# Autodesk Inventor assembly: Sestava
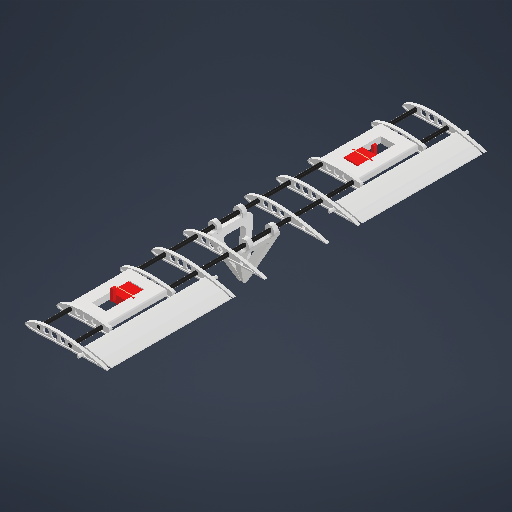
[picture p0: Inventor's stored thumbnail of the model, 512x512]
Saved by Autodesk Inventor 2026 (Build 300175050, 175E)
## iProperties
Created: 2026-02-21
Part Number: Sestava
Document SubType Name: Assembly
Designer: marti
Mass: 312.301 g
Surface Area: 1695.85 cm^2
Volume: 283.461 cm^3
Density: 1.10174 g/cm^3
Author: marti
## Documents named in this file (9)
- F:\Ročníkovka\RP_Svitek\3d model\lepší\Sestava.iam
- F:\Ročníkovka\RP_Svitek\3d model\lepší\tyč.ipt
- F:\Ročníkovka\RP_Svitek\3d model\lepší\Profil.ipt
- F:\Ročníkovka\RP_Svitek\3d model\lepší\NOAileron.ipt
- F:\Ročníkovka\RP_Svitek\3d model\lepší\Aileronn.ipt
- F:\Ročníkovka\RP_Svitek\3d model\lepší\vetrovaniig.ipt
- F:\Ročníkovka\RP_Svitek\3d model\lepší\trojúhleník.ipt
- F:\Ročníkovka\RP_Svitek\3d model\lepší\SERVO držák.ipt
- F:\Ročníkovka\RP_Svitek\3d model\lepší\Servo.ipt
## Components (21 placed, 8 different names)
1. tyč:1 — Proti sobě:1, Stejný směr:1, Proti sobě:2, Proti sobě:3, Proti sobě:4, Proti sobě:8, Proti sobě:10, Proti sobě:12, Proti sobě:14, Proti sobě:17, Stejný směr:2, Proti sobě:22, Proti sobě:27, Proti sobě:29, Proti sobě:31, Proti sobě:43, Proti sobě:47, Proti sobě:53, Proti sobě:54
2. tyč:2 — Proti sobě:4, Proti sobě:5, Proti sobě:6, Proti sobě:7, Proti sobě:9, Proti sobě:11, Proti sobě:13, Proti sobě:15, Proti sobě:18, Stejný směr:2, Stejný směr:3, Proti sobě:23, Stejný směr:4, Proti sobě:28, Proti sobě:30, Proti sobě:32, Proti sobě:44, Proti sobě:46, Proti sobě:51, Stejný směr:14
3. Profil:1 — Proti sobě:2, Proti sobě:6, Stejný směr:4, Proti sobě:24, Proti sobě:25, Stejný směr:5
4. Profil:2 — Proti sobě:3, Proti sobě:7, Proti sobě:16, Proti sobě:19, Proti sobě:20, Stejný směr:3, Stejný směr:9
5. NOAileron:1 — Proti sobě:8, Proti sobě:9, Stejný směr:5, Stejný směr:6
6. NOAileron:2 — Proti sobě:10, Proti sobě:11, Stejný směr:6, Stejný směr:7, Proti sobě:45
7. NOAileron:3 — Proti sobě:14, Proti sobě:15, Stejný směr:9, Stejný směr:10
8. NOAileron:4 — Proti sobě:12, Proti sobě:13, Stejný směr:10, Stejný směr:11, Proti sobě:48
9. Profil:3 — Proti sobě:22, Proti sobě:23, Proti sobě:26, Stejný směr:7, Stejný směr:8
10. Profil:4 — Proti sobě:17, Proti sobě:18, Proti sobě:21, Stejný směr:11, Stejný směr:12
11. Aileronn:1 — Proti sobě:16, Proti sobě:19, Proti sobě:20, Proti sobě:21
12. Aileronn:2 — Proti sobě:24, Proti sobě:25, Proti sobě:26
13. Profil:5 — Proti sobě:27, Proti sobě:28, Stejný směr:8
14. Profil:6 — Proti sobě:29, Proti sobě:30, Stejný směr:12, Stejný směr:13
15. vetrovaniig:1 — Proti sobě:31, Proti sobě:32, Stejný směr:13
16. SERVO držák:1 — Proti sobě:41, Proti sobě:42, Proti sobě:43, Proti sobě:44, Proti sobě:45
17. Servo:1 — Proti sobě:41, Proti sobě:42
18. SERVO držák:2 — Proti sobě:46, Proti sobě:47, Proti sobě:48, Proti sobě:49, Proti sobě:50
19. Servo:2 — Proti sobě:49, Proti sobě:50
20. trojúhleník:1 — Proti sobě:51, Stejný směr:14, Proti sobě:55
21. trojúhleník:2 — Proti sobě:53, Proti sobě:54, Proti sobě:55
## Relationships (60: Mate 46, Flush 14)
- Proti sobě:1 [Mate]: tyč:1
- Stejný směr:1 [Flush]: tyč:1
- Proti sobě:2 [Mate]: tyč:1 ↔ Profil:1
- Proti sobě:3 [Mate]: tyč:1 ↔ Profil:2
- Proti sobě:4 [Mate] (-50 mm): tyč:1 ↔ tyč:2
- Proti sobě:5 [Mate]: tyč:2
- Proti sobě:6 [Mate]: tyč:2 ↔ Profil:1
- Proti sobě:7 [Mate]: tyč:2 ↔ Profil:2
- Proti sobě:8 [Mate]: tyč:1 ↔ NOAileron:1
- Proti sobě:9 [Mate]: tyč:2 ↔ NOAileron:1
- Proti sobě:10 [Mate]: tyč:1 ↔ NOAileron:2
- Proti sobě:11 [Mate]: tyč:2 ↔ NOAileron:2
- Proti sobě:12 [Mate]: tyč:1 ↔ NOAileron:4
- Proti sobě:13 [Mate]: tyč:2 ↔ NOAileron:4
- Proti sobě:14 [Mate]: tyč:1 ↔ NOAileron:3
- Proti sobě:15 [Mate]: tyč:2 ↔ NOAileron:3
- Proti sobě:16 [Mate]: Profil:2 ↔ Aileronn:1
- Proti sobě:17 [Mate]: tyč:1 ↔ Profil:4
- Proti sobě:18 [Mate]: tyč:2 ↔ Profil:4
- Proti sobě:19 [Mate]: Profil:2 ↔ Aileronn:1
- Proti sobě:20 [Mate] (2 mm): Profil:2 ↔ Aileronn:1
- Stejný směr:2 [Flush]: tyč:1 ↔ tyč:2
- Stejný směr:3 [Flush]: tyč:2 ↔ Profil:2
- Proti sobě:21 [Mate] (2 mm): Profil:4 ↔ Aileronn:1
- Proti sobě:22 [Mate]: tyč:1 ↔ Profil:3
- Proti sobě:23 [Mate]: tyč:2 ↔ Profil:3
- Stejný směr:4 [Flush]: tyč:2 ↔ Profil:1
- Proti sobě:24 [Mate]: Profil:1 ↔ Aileronn:2
- Proti sobě:25 [Mate] (2 mm): Profil:1 ↔ Aileronn:2
- Proti sobě:26 [Mate] (2 mm): Profil:3 ↔ Aileronn:2
- Proti sobě:27 [Mate]: tyč:1 ↔ Profil:5
- Proti sobě:28 [Mate]: tyč:2 ↔ Profil:5
- Proti sobě:29 [Mate]: tyč:1 ↔ Profil:6
- Proti sobě:30 [Mate]: tyč:2 ↔ Profil:6
- Stejný směr:5 [Flush] (50 mm): Profil:1 ↔ NOAileron:1
- Stejný směr:6 [Flush] (-100 mm): NOAileron:1 ↔ NOAileron:2
- Stejný směr:7 [Flush] (-50 mm): NOAileron:2 ↔ Profil:3
- Stejný směr:8 [Flush] (50 mm): Profil:3 ↔ Profil:5
- Stejný směr:9 [Flush] (50 mm): Profil:2 ↔ NOAileron:3
- Stejný směr:10 [Flush] (100 mm): NOAileron:3 ↔ NOAileron:4
- Stejný směr:11 [Flush] (50 mm): NOAileron:4 ↔ Profil:4
- Stejný směr:12 [Flush] (50 mm): Profil:4 ↔ Profil:6
- Proti sobě:31 [Mate]: tyč:1 ↔ vetrovaniig:1
- Proti sobě:32 [Mate]: tyč:2 ↔ vetrovaniig:1
- Stejný směr:13 [Flush] (-48 mm): Profil:6 ↔ vetrovaniig:1
- Proti sobě:41 [Mate]: SERVO držák:1 ↔ Servo:1
- Proti sobě:42 [Mate]: SERVO držák:1 ↔ Servo:1
- Proti sobě:43 [Mate]: tyč:1 ↔ SERVO držák:1
- Proti sobě:44 [Mate]: tyč:2 ↔ SERVO držák:1
- Proti sobě:45 [Mate]: NOAileron:2 ↔ SERVO držák:1
- Proti sobě:46 [Mate]: tyč:2 ↔ SERVO držák:2
- Proti sobě:47 [Mate]: tyč:1 ↔ SERVO držák:2
- Proti sobě:48 [Mate]: NOAileron:4 ↔ SERVO držák:2
- Proti sobě:49 [Mate]: SERVO držák:2 ↔ Servo:2
- Proti sobě:50 [Mate]: SERVO držák:2 ↔ Servo:2
- Proti sobě:51 [Mate]: tyč:2 ↔ trojúhleník:1
- Stejný směr:14 [Flush] (300 mm): tyč:2 ↔ trojúhleník:1
- Proti sobě:53 [Mate]: tyč:1 ↔ trojúhleník:2
- Proti sobě:54 [Mate] (-300 mm): tyč:1 ↔ trojúhleník:2
- Proti sobě:55 [Mate]: trojúhleník:1 ↔ trojúhleník:2
